# Autodesk Inventor assembly: Ensamblaje pedal
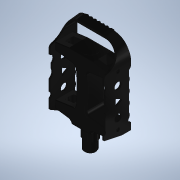
[picture p0: Inventor's stored thumbnail of the model, 180x180]
Saved by Autodesk Inventor 2021 (Build 250183000, 183)
## iProperties
Created: 2020-11-11
Part Number: Ensamblaje pedal
Description: STEP AP214
Document SubType Name: Assembly
Designer: j2seb
Sending System: SolidWorks 2017
Preprocessor: SwSTEP 2.0
Title: Ensamblaje pedal.STEP
Revision Number: ANY
## Documents named in this file (4)
- C:\Users\leo7s\Documents\Universidad\03 APM\04 Gitrespository\Proyecto_APM\02 Inventor\Ensamblaje pedal.iam
- C:\Users\leo7s\Documents\Universidad\03 APM\04 Gitrespository\Proyecto_APM\02 Inventor\Pedal.ipt
- C:\Users\leo7s\Documents\Universidad\03 APM\04 Gitrespository\Proyecto_APM\02 Inventor\Perno pedal.ipt
- C:\Users\leo7s\Documents\Universidad\03 APM\04 Gitrespository\Proyecto_APM\02 Inventor\Tapa pedal.ipt
## Components (3 placed, 3 different names)
1. Pedal_1 — Coincidencia:1, Coincidencia:2
2. Perno pedal_2 — Coincidencia:1, Coincidencia:2
3. Tapa pedal_3
## Relationships (2: Mate 2)
- Coincidencia:1 [Mate]: Pedal_1 ↔ Perno pedal_2
- Coincidencia:2 [Mate]: Pedal_1 ↔ Perno pedal_2
